# Autodesk Inventor assembly: GE-12071
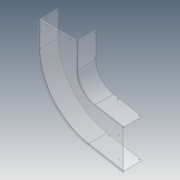
[picture p0: Inventor's stored thumbnail of the model, 180x180]
Saved by Autodesk Inventor 2012 (Build 160160000, 160)
## iProperties
Created: 2011-09-22
Part Number: GE-12071
Document SubType Name: Assembly
Designer: dfoster
Author: dfoster
## Documents named in this file (4)
- C:\Data Folder\FRC 2012 Field\Components\GE-12071.iam
- C:\Data Folder\FRC 2012 Field\Components\GE-12071-01.ipt
- C:\Data Folder\FRC 2012 Field\Components\GE-12071-02.ipt
- C:\Data Folder\FRC 2012 Field\Components\GE-12071-03.ipt
## Components (3 placed, 3 different names)
1. GE-12071-01:1 — Flush:1, Flush:2
2. GE-12071-02:1 — Flush:1
3. GE-12071-03:1 — Flush:2
## Relationships (2: Flush 2)
- Flush:1: GE-12071-01:1 ↔ GE-12071-02:1
- Flush:2: GE-12071-01:1 ↔ GE-12071-03:1
